# Autodesk Inventor assembly: MainAssy
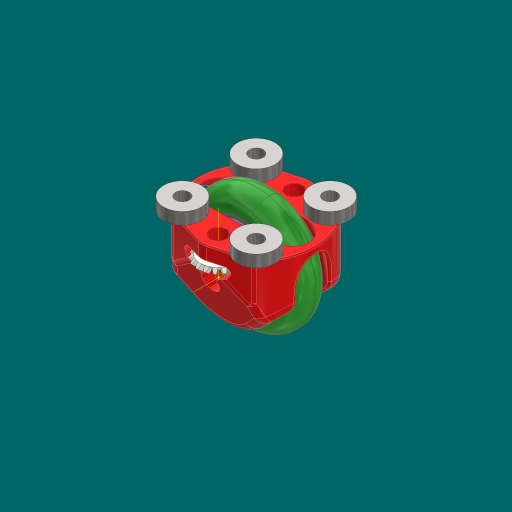
[picture p0: Inventor's stored thumbnail of the model, 512x512]
Saved by Autodesk Inventor 2023.1 (Build 271208000, 208)
## iProperties
Created: 2022-09-24
Part Number: MainAssy
Document SubType Name: Assembly
Designer: zac-h
Author: zac-h
## Documents named in this file (7)
- C:\Users\zac-h\Documents\CAD\guardSwerve3\MainAssy.iam
- C:\Users\zac-h\Documents\CAD\guardSwerve3\carriage.ipt
- C:\Users\zac-h\Documents\CAD\guardSwerve3\MainAssy\Design Accelerator\Bevel Gears1.iam
- C:\Users\zac-h\Documents\CAD\VEX-CAD-Inventor-1.3.0\VEX-CAD-Inventor-1.3.0\Motion\Wheels\Tractions\2.75 Traction, Square.ipt
- C:\Users\zac-h\Documents\CAD\VEX-CAD-Inventor-1.3.0\VEX-CAD-Inventor-1.3.0\Motion\Spacers\Washer Teflon\TWasher .375 OD x .04000.ipt
- C:\Users\zac-h\Documents\CAD\VEX-CAD-Inventor-1.3.0\VEX-CAD-Inventor-1.3.0\Motion\Spacers\Washer Teflon.ipt
- C:\Users\zac-h\Documents\CAD\guardSwerve3\bearing.ipt
## Components (11 placed, 5 different names)
1. carriage:1 — Mate:1, Angle:1, Mate:2, Mate:3, Insert:1, Insert:2, Insert:3, Insert:4
2. Bevel Gears:1 [sub-assembly] — Mate:1, Angle:1, Mate:2
3. 2.75 Traction, Square:1 — Mate:3, Mate:4
4. TWasher .375 OD x .04000:1 — Insert:1, Flush:1
5. TWasher .375 OD x .04000:2 — Insert:4
6. TWasher .375 OD x .04000:3 — Insert:2
7. TWasher .375 OD x .04000:4 — Insert:3
8. bearing:1 — Flush:1
9. bearing:2
10. bearing:3
11. bearing:4
## Component patterns: (4 elements, first: bearing:1)
## Relationships (10: Mate 4, Insert 4, Angle 1, Flush 1)
- Mate:1: carriage:1 ↔ Bevel Gears:1
- Angle:1 (0 deg): carriage:1 ↔ Bevel Gears:1
- Mate:2: carriage:1 ↔ Bevel Gears:1
- Mate:3: carriage:1 ↔ 2.75 Traction, Square:1
- Mate:4: 2.75 Traction, Square:1
- Insert:1: carriage:1 ↔ TWasher .375 OD x .04000:1
- Insert:2: carriage:1 ↔ TWasher .375 OD x .04000:3
- Insert:3: carriage:1 ↔ TWasher .375 OD x .04000:4
- Insert:4: carriage:1 ↔ TWasher .375 OD x .04000:2
- Flush:1: TWasher .375 OD x .04000:1 ↔ bearing:1
